# Autodesk Inventor assembly: Lagerhalterung
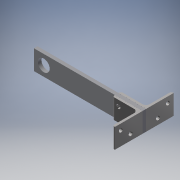
[picture p0: Inventor's stored thumbnail of the model, 180x180]
Saved by Autodesk Inventor 2018 (Build 220112000, 112)
## iProperties
Created: 2018-01-29
Part Number: Lagerhalterung
Material: Generisch
Document SubType Name: Assembly
Designer: Julian
Author: Julian
## Documents named in this file (3)
- C:\Users\Julian\Desktop\Schule\5AHME\Diplomarbeit\Git\fuettr_prototype\Mechanical\Inventorskizzen\Lagerhalterung.iam
- C:\Users\Julian\Desktop\Schule\5AHME\Diplomarbeit\Git\fuettr_prototype\Mechanical\Inventorskizzen\ISO 657-1 - L70x70x6-50.ipt
- C:\Users\Julian\Desktop\Schule\5AHME\Diplomarbeit\Git\fuettr_prototype\Mechanical\Inventorskizzen\Lagerstuetze.ipt
## Components (3 placed, 2 different names)
1. ISO 657-1 - L70x70x6-50:1 — Starr:1
2. ISO 657-1 - L70x70x6-50:2 — Starr:2
3. Lagerstuetze:1 — Starr:1, Starr:2
## Relationships (2: WeldJoint 2)
- Starr:1 [WeldJoint]: ISO 657-1 - L70x70x6-50:1 ↔ Lagerstuetze:1
- Starr:2 [WeldJoint]: ISO 657-1 - L70x70x6-50:2 ↔ Lagerstuetze:1
